# Autodesk Inventor assembly: Forearm2
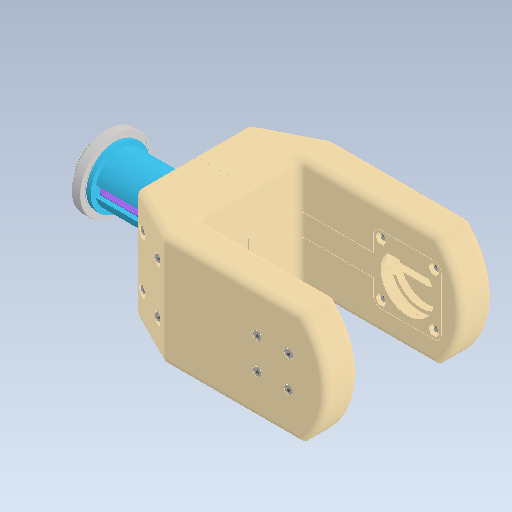
[picture p0: Inventor's stored thumbnail of the model, 512x512]
Saved by Autodesk Inventor 2021 (Build 250183000, 183)
## iProperties
Created: 2020-03-07
Part Number: Forearm2
Document SubType Name: Assembly
Designer: JochenAlt
Author: JochenAlt
## Documents named in this file (7)
- C:\Users\Jochen Alt\Documents\Daten\Projects\MiniBot\CAD\Forearm.iam
- C:\Users\Jochen Alt\Documents\Daten\Projects\MiniBot\CAD\Forearm.ipt
- C:\Users\Jochen Alt\Documents\Daten\Projects\MiniBot\CAD\ForearmShaft.ipt
- C:\Users\Jochen Alt\Documents\Daten\Projects\MiniBot\CAD\extern\bearings\25x32x4\W 61705-2RS1.iam
- C:\Users\Jochen Alt\Documents\Daten\Projects\MiniBot\CAD\extern\accessories\Hex Spacer 10mm.ipt
- D:\Projects\MiniBot\CAD\extern\DIN 912\DIN 912 - M2 x 0.4 x 12 x 11.ipt
- D:\Projects\MiniBot\CAD\extern\DIN 912\DIN 912 - M2 x 0.4 x 20 x 19.ipt
## Components (31 placed, 6 different names)
1. Forearm:1 — Passend:2, Insert:1, Insert:2, Insert:3, Insert:4, Insert:5, Insert:6, Insert:7, Insert:8, Insert:9, Insert:10, Insert:11, Insert:12, Insert:13, Insert:14, Insert:15, Insert:16, Passend:12, Passend:13, Passend:14, Passend:15, Winkel:1, Fluchtend:1
2. ForearmShaft:1 — Passend:2, Passend:3, Passend:4, Passend:5, Passend:6, Mate:8, Mate:9, Mate:10, Mate:11, Passend:26, Passend:27, Passend:29, Winkel:1, Fluchtend:1, Passend:32, Passend:34
3. W 61705-2RS1:1 [sub-assembly] — Passend:3, Passend:5
4. W 61705-2RS1:2 [sub-assembly] — Passend:4, Passend:6
5. DIN 912 - replaced by DIN EN ISO 4762 M2 x 12:1 — Insert:1
6. DIN 912 - replaced by DIN EN ISO 4762 M2 x 12:2 — Insert:2
7. DIN 912 - replaced by DIN EN ISO 4762 M2 x 12:3 — Insert:3
8. DIN 912 - replaced by DIN EN ISO 4762 M2 x 12:4 — Insert:4
9. DIN 912 - replaced by DIN EN ISO 4762 M2 x 20:1 — Insert:5
10. DIN 912 - replaced by DIN EN ISO 4762 M2 x 20:2 — Insert:6
11. DIN 912 - replaced by DIN EN ISO 4762 M2 x 20:3 — Insert:7
12. DIN 912 - replaced by DIN EN ISO 4762 M2 x 20:4 — Insert:8
13. DIN 912 - replaced by DIN EN ISO 4762 M2 x 12:5 — Insert:9
14. DIN 912 - replaced by DIN EN ISO 4762 M2 x 12:6 — Insert:10, Passend:31
15. DIN 912 - replaced by DIN EN ISO 4762 M2 x 20:5 — Insert:11
16. DIN 912 - replaced by DIN EN ISO 4762 M2 x 20:6 — Insert:12
17. DIN 912 - replaced by DIN EN ISO 4762 M2 x 20:7 — Insert:13, Passend:33
18. DIN 912 - replaced by DIN EN ISO 4762 M2 x 20:8 — Insert:14
19. DIN 912 - replaced by DIN EN ISO 4762 M2 x 12:7 — Insert:15
20. DIN 912 - replaced by DIN EN ISO 4762 M2 x 12:8 — Insert:16
21. W 61705-2RS1:3 [sub-assembly] — Mate:8, Mate:11
22. W 61705-2RS1:4 [sub-assembly] — Mate:9, Mate:10
23. Hex Spacer 10mm:2 — Passend:12
24. Hex Spacer 10mm:1 — Passend:13, Passend:19, Passend:20, Passend:29
25. Hex Spacer 10mm:3 — Passend:14, Passend:18, Passend:24
26. Hex Spacer 10mm:4 — Passend:15, Passend:16, Passend:26, Passend:30
27. Hex Spacer 10mm:6 — Passend:16, Passend:30
28. Hex Spacer 10mm:7 — Passend:19, Passend:20
29. Hex Spacer 10mm:8 — Passend:18, Passend:24, Passend:27
30. Hex Spacer 10mm:9 — Passend:31, Passend:32
31. Hex Spacer 10mm:10 — Passend:33, Passend:34
## Relationships (44: Mate 26, Insert 16, Angle 1, Flush 1)
- Passend:2 [Mate]: Forearm:1 ↔ ForearmShaft:1
- Passend:3 [Mate]: ForearmShaft:1 ↔ W 61705-2RS1:1
- Passend:4 [Mate]: ForearmShaft:1 ↔ W 61705-2RS1:2
- Passend:5 [Mate]: ForearmShaft:1 ↔ W 61705-2RS1:1
- Passend:6 [Mate]: ForearmShaft:1 ↔ W 61705-2RS1:2
- Insert:1: Forearm:1 ↔ DIN 912 - replaced by DIN EN ISO 4762 M2 x 12:1
- Insert:2: Forearm:1 ↔ DIN 912 - replaced by DIN EN ISO 4762 M2 x 12:2
- Insert:3: Forearm:1 ↔ DIN 912 - replaced by DIN EN ISO 4762 M2 x 12:3
- Insert:4: Forearm:1 ↔ DIN 912 - replaced by DIN EN ISO 4762 M2 x 12:4
- Insert:5: Forearm:1 ↔ DIN 912 - replaced by DIN EN ISO 4762 M2 x 20:1
- Insert:6: Forearm:1 ↔ DIN 912 - replaced by DIN EN ISO 4762 M2 x 20:2
- Insert:7: Forearm:1 ↔ DIN 912 - replaced by DIN EN ISO 4762 M2 x 20:3
- Insert:8: Forearm:1 ↔ DIN 912 - replaced by DIN EN ISO 4762 M2 x 20:4
- Insert:9: Forearm:1 ↔ DIN 912 - replaced by DIN EN ISO 4762 M2 x 12:5
- Insert:10: Forearm:1 ↔ DIN 912 - replaced by DIN EN ISO 4762 M2 x 12:6
- Insert:11: Forearm:1 ↔ DIN 912 - replaced by DIN EN ISO 4762 M2 x 20:5
- Insert:12: Forearm:1 ↔ DIN 912 - replaced by DIN EN ISO 4762 M2 x 20:6
- Insert:13: Forearm:1 ↔ DIN 912 - replaced by DIN EN ISO 4762 M2 x 20:7
- Insert:14: Forearm:1 ↔ DIN 912 - replaced by DIN EN ISO 4762 M2 x 20:8
- Insert:15: Forearm:1 ↔ DIN 912 - replaced by DIN EN ISO 4762 M2 x 12:7
- Insert:16: Forearm:1 ↔ DIN 912 - replaced by DIN EN ISO 4762 M2 x 12:8
- Mate:8: ForearmShaft:1 ↔ W 61705-2RS1:3
- Mate:9: ForearmShaft:1 ↔ W 61705-2RS1:4
- Mate:10: ForearmShaft:1 ↔ W 61705-2RS1:4
- Mate:11: ForearmShaft:1 ↔ W 61705-2RS1:3
- Passend:12 [Mate]: Forearm:1 ↔ Hex Spacer 10mm:2
- Passend:13 [Mate]: Forearm:1 ↔ Hex Spacer 10mm:1
- Passend:14 [Mate]: Forearm:1 ↔ Hex Spacer 10mm:3
- Passend:15 [Mate]: Forearm:1 ↔ Hex Spacer 10mm:4
- Passend:16 [Mate]: Hex Spacer 10mm:4 ↔ Hex Spacer 10mm:6
- Passend:18 [Mate]: Hex Spacer 10mm:3 ↔ Hex Spacer 10mm:8
- Passend:19 [Mate]: Hex Spacer 10mm:1 ↔ Hex Spacer 10mm:7
- Passend:20 [Mate] (10 mm): Hex Spacer 10mm:1 ↔ Hex Spacer 10mm:7
- Passend:24 [Mate] (10 mm): Hex Spacer 10mm:3 ↔ Hex Spacer 10mm:8
- Passend:26 [Mate]: ForearmShaft:1 ↔ Hex Spacer 10mm:4
- Passend:27 [Mate]: ForearmShaft:1 ↔ Hex Spacer 10mm:8
- Passend:29 [Mate]: ForearmShaft:1 ↔ Hex Spacer 10mm:1
- Passend:30 [Mate] (10 mm): Hex Spacer 10mm:4 ↔ Hex Spacer 10mm:6
- Winkel:1 [Angle] (0 deg): Forearm:1 ↔ ForearmShaft:1
- Fluchtend:1 [Flush]: Forearm:1 ↔ ForearmShaft:1
- Passend:31 [Mate]: DIN 912 - replaced by DIN EN ISO 4762 M2 x 12:6 ↔ Hex Spacer 10mm:9
- Passend:32 [Mate]: ForearmShaft:1 ↔ Hex Spacer 10mm:9
- Passend:33 [Mate]: DIN 912 - replaced by DIN EN ISO 4762 M2 x 20:7 ↔ Hex Spacer 10mm:10
- Passend:34 [Mate]: ForearmShaft:1 ↔ Hex Spacer 10mm:10
